# Autodesk Inventor assembly: Assembly
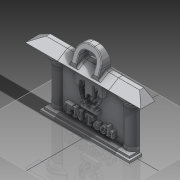
[picture p0: Inventor's stored thumbnail of the model, 180x180]
Saved by Autodesk Inventor 2018 (Build 220112000, 112)
## iProperties
Created: 2017-12-11
Part Number: Assembly
Document SubType Name: Assembly
Designer: Rus
Author: Rus
## Documents named in this file (9)
- F:\2017 TN Tech Ornament\Shrink ASM\Assembly.iam
- F:\2017 TN Tech Ornament\Shrink ASM\Shrink ASM RightP.ipt
- F:\2017 TN Tech Ornament\Shrink ASM\Shrink ASM Top.ipt
- F:\2017 TN Tech Ornament\Shrink ASM\Shrink ASM Logo.ipt
- F:\2017 TN Tech Ornament\Shrink ASM\Shrink ASM Left Pillar.ipt
- F:\2017 TN Tech Ornament\Shrink ASM\Shrink ASM RightP Bot.ipt
- F:\2017 TN Tech Ornament\Shrink ASM\Shrink ASM Left Pillar Bot.ipt
- F:\2017 TN Tech Ornament\Shrink ASM\New Bot.ipt
- F:\2017 TN Tech Ornament\Shrink ASM\Bad PillarS.ipt
## Components (8 placed, 8 different names)
1. Shrink ASM RightP:1 — Flush:4, Mate:3, Tangent:2, Flush:9, Angle:5, Flush:19, Flush:21, Mate:12
2. Shrink ASM Top:1 — Flush:5, Mate:5, Mate:6, Angle:1, Flush:15, Flush:18
3. Shrink ASM Logo:1 — Flush:4, Flush:5, Mate:2, Mate:3, Mate:5, Mate:7, Angle:2, Flush:16, Flush:17, Flush:18, Flush:19, Flush:20, Mate:12
4. Shrink ASM Left Pillar:1 — Mate:2, Tangent:1, Flush:20, Flush:21, Flush:22
5. Shrink ASM RightP Bot:1 — Tangent:2, Flush:9, Angle:5, Flush:13, Flush:14, Flush:16
6. Shrink ASM Left Pillar Bot:1 — Tangent:1, Flush:13, Flush:14, Flush:15, Flush:17, Flush:23
7. New Bot:1 — Flush:22
8. Bad PillarS:1 — Flush:23
## Relationships (28: Flush 14, Mate 9, Angle 3, Tangent 2)
- Flush:4: Shrink ASM RightP:1 ↔ Shrink ASM Logo:1
- Flush:5: Shrink ASM Top:1 ↔ Shrink ASM Logo:1
- Mate:2: Shrink ASM Logo:1 ↔ Shrink ASM Left Pillar:1
- Mate:3: Shrink ASM RightP:1 ↔ Shrink ASM Logo:1
- Mate:5: Shrink ASM Top:1 ↔ Shrink ASM Logo:1
- Mate:6: Shrink ASM Top:1
- Angle:1 (0 deg): Shrink ASM Top:1
- Mate:7: Shrink ASM Logo:1
- Angle:2 (0 deg): Shrink ASM Logo:1
- Mate:8
- Mate:10
- Mate:11
- Tangent:1: Shrink ASM Left Pillar:1 ↔ Shrink ASM Left Pillar Bot:1
- Tangent:2: Shrink ASM RightP:1 ↔ Shrink ASM RightP Bot:1
- Flush:9: Shrink ASM RightP:1 ↔ Shrink ASM RightP Bot:1
- Angle:5 (0 deg): Shrink ASM RightP:1 ↔ Shrink ASM RightP Bot:1
- Flush:13: Shrink ASM RightP Bot:1 ↔ Shrink ASM Left Pillar Bot:1
- Flush:14: Shrink ASM RightP Bot:1 ↔ Shrink ASM Left Pillar Bot:1
- Flush:15: Shrink ASM Top:1 ↔ Shrink ASM Left Pillar Bot:1
- Flush:16: Shrink ASM Logo:1 ↔ Shrink ASM RightP Bot:1
- Flush:17: Shrink ASM Logo:1 ↔ Shrink ASM Left Pillar Bot:1
- Flush:18: Shrink ASM Top:1 ↔ Shrink ASM Logo:1
- Flush:19: Shrink ASM RightP:1 ↔ Shrink ASM Logo:1
- Flush:20: Shrink ASM Logo:1 ↔ Shrink ASM Left Pillar:1
- Flush:21: Shrink ASM RightP:1 ↔ Shrink ASM Left Pillar:1
- Mate:12: Shrink ASM RightP:1 ↔ Shrink ASM Logo:1
- Flush:22: Shrink ASM Left Pillar:1 ↔ New Bot:1
- Flush:23: Shrink ASM Left Pillar Bot:1 ↔ Bad PillarS:1
